# Autodesk Inventor assembly: FULL FINGE6
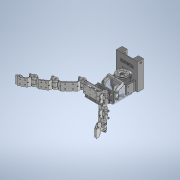
[picture p0: Inventor's stored thumbnail of the model, 180x180]
Saved by Autodesk Inventor 2021 (Build 250183000, 183)
## iProperties
Created: 2022-10-03
Part Number: FULL FINGE6
Document SubType Name: Assembly
Designer: ereg140
Author: ereg140
## Documents named in this file (10)
- \\files.auckland.ac.nz\myhome\Documents\GitHub\hand\FULL FINGE7.iam
- \\files.auckland.ac.nz\myhome\Documents\GitHub\hand\XM430 Motor\XM430-Working-Shaft.iam
- \\files.auckland.ac.nz\myhome\Documents\GitHub\hand\Pully_smlaller.ipt
- \\files.auckland.ac.nz\myhome\Documents\GitHub\hand\Dovetail\dovetail_female_Dyna_Mount.ipt
- \\files.auckland.ac.nz\myhome\Documents\GitHub\hand\Dynamixel_Palm_Bracket_2.ipt
- \\files.auckland.ac.nz\myhome\Documents\GitHub\hand\Tendon_Center.ipt
- \\files.auckland.ac.nz\myhome\Documents\GitHub\hand\PLANGE7\Phalalnge7_HDM_45mm.ipt
- \\files.auckland.ac.nz\myhome\Documents\GitHub\hand\PLANGE7\Phalalnge7_HDM_35mm.ipt
- \\files.auckland.ac.nz\myhome\Documents\GitHub\hand\PLANGE7\Phalalnge7_35mm_TIP_hdm.ipt
- \\files.auckland.ac.nz\myhome\Documents\GitHub\hand\PLANGE7\FINGIE_7_palm_50mm.ipt
## Components (12 placed, 9 different names)
1. XM430-Working-Shaft:1 [sub-assembly] — Angle:1, Rigid:4, Mate:1, Mate:2, Slider:1, Rigid:7, Rigid:8
2. Pully_smlaller:1 — Rigid:4
3. dovetail_female_Dyna_Mount:1 — Mate:1, Mate:2, Slider:1
4. Dynamixel_Palm_Bracket_2:1 — Rigid:7, Rigid:9
5. Tendon_Center:1 — Rigid:8
6. FINGIE_7_palm_50mm:1 — Rigid:9, Planar:4, Cylindrical:7, Cylindrical:12, Planar:9
7. Phalalnge7_35mm_TIP_hdm:2 — Planar:6, Cylindrical:9
8. Phalalnge7_HDM_35mm:2 — Planar:5, Planar:6, Cylindrical:8, Cylindrical:9
9. Phalalnge7_HDM_45mm:2 — Planar:4, Planar:5, Cylindrical:7, Cylindrical:8
10. Phalalnge7_35mm_TIP_hdm:3 — Cylindrical:11
11. Phalalnge7_HDM_35mm:3 — Cylindrical:10, Cylindrical:11
12. Phalalnge7_HDM_45mm:3 — Cylindrical:10, Cylindrical:12, Planar:9
## Relationships (20: PlanarJoint 6, CylindricalJoint 6, WeldJoint 4, Mate 2, Angle 1, TranslationJoint 1)
- Angle:1 (0 deg): XM430-Working-Shaft:1
- Rigid:4 [WeldJoint]: XM430-Working-Shaft:1 ↔ Pully_smlaller:1
- Mate:1: XM430-Working-Shaft:1 ↔ dovetail_female_Dyna_Mount:1
- Mate:2: XM430-Working-Shaft:1 ↔ dovetail_female_Dyna_Mount:1
- Slider:1 [TranslationJoint]: XM430-Working-Shaft:1 ↔ dovetail_female_Dyna_Mount:1
- Rigid:7 [WeldJoint]: XM430-Working-Shaft:1 ↔ Dynamixel_Palm_Bracket_2:1
- Rigid:8 [WeldJoint]: XM430-Working-Shaft:1 ↔ Tendon_Center:1
- Rigid:9 [WeldJoint]: Dynamixel_Palm_Bracket_2:1 ↔ FINGIE_7_palm_50mm:1
- Planar:4: FINGIE_7_palm_50mm:1 ↔ Phalalnge7_HDM_45mm:2
- Planar:5: Phalalnge7_HDM_35mm:2 ↔ Phalalnge7_HDM_45mm:2
- Planar:6: Phalalnge7_35mm_TIP_hdm:2 ↔ Phalalnge7_HDM_35mm:2
- Cylindrical:7: FINGIE_7_palm_50mm:1 ↔ Phalalnge7_HDM_45mm:2
- Cylindrical:8: Phalalnge7_HDM_35mm:2 ↔ Phalalnge7_HDM_45mm:2
- Cylindrical:9: Phalalnge7_35mm_TIP_hdm:2 ↔ Phalalnge7_HDM_35mm:2
- [PlanarJoint]: Phalalnge7_HDM_35mm:3 ↔ Phalalnge7_HDM_45mm:3
- [PlanarJoint]: Phalalnge7_35mm_TIP_hdm:3 ↔ Phalalnge7_HDM_35mm:3
- Cylindrical:10: Phalalnge7_HDM_35mm:3 ↔ Phalalnge7_HDM_45mm:3
- Cylindrical:11: Phalalnge7_35mm_TIP_hdm:3 ↔ Phalalnge7_HDM_35mm:3
- Cylindrical:12: FINGIE_7_palm_50mm:1 ↔ Phalalnge7_HDM_45mm:3
- Planar:9: FINGIE_7_palm_50mm:1 ↔ Phalalnge7_HDM_45mm:3
## Named parameters: sa_0 = 30000, d48_d34 = 0 mm, d49_d35 = 0 mm, d50_d44 = 179.657847 deg, d51_d45 = -0.5 mm, d52_d46 = 147.937676 deg, d53_d47 = 0.5 mm
note: some values were not read from the file. Shown as the stored number, unit unknown: "sa_0".
